# Autodesk Inventor assembly: AirtightAftSectionAssembly0
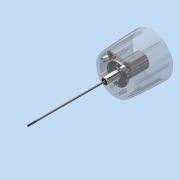
[picture p0: Inventor's stored thumbnail of the model, 180x180]
Saved by Autodesk Inventor 2017 (Build 210142000, 142)
## iProperties
Created: 2016-10-23
Part Number: AirtightAftSectionAssembly0
Document SubType Name: Assembly
Designer: techn
Author: techn
## Documents named in this file (6)
- D:\OneDrive\Documents\Other Projects\Submarine\CAD\aft\AirtightAftSectionAssembly0.iam
- D:\OneDrive\Documents\Other Projects\Submarine\CAD\aft\MotorAssembly0.iam
- D:\OneDrive\Documents\Other Projects\Submarine\CAD\aft\AftSectionAirtightRear.ipt
- D:\OneDrive\Documents\Other Projects\Submarine\CAD\common\PushRodSeal\Engel3mm\Engel3mmAssembly.iam
- D:\OneDrive\Documents\Other Projects\Submarine\CAD\common\PushRodSeal\bearingHousing.ipt
- D:\OneDrive\Documents\Other Projects\Submarine\CAD\common\SleeveBearing3mmFlanged.ipt
## Components (8 placed, 5 different names)
1. MotorAssembly0:1 [sub-assembly] — Mate:5, Mate:6, Mate:7
2. AftSectionAirtightRear:1 — Mate:5, Mate:6, Mate:7, Mate:23, Mate:24, Angle:1, Angle:2, Mate:25, Mate:26, Mate:33, Mate:34, Mate:35, Mate:36
3. Engel3mmAssembly:1 [sub-assembly] — Mate:23, Angle:2, Mate:25, Mate:31
4. Engel3mmAssembly:2 [sub-assembly] — Mate:24, Angle:1, Mate:26, Mate:32
5. bearingHousing:1 — Mate:27, Mate:28, Mate:33, Mate:34
6. bearingHousing:2 — Mate:29, Mate:30, Mate:31, Mate:35, Mate:36
7. SleeveBearing3mmFlanged:1 — Mate:27, Mate:28, Mate:32
8. SleeveBearing3mmFlanged:2 — Mate:29, Mate:30
## Relationships (19: Mate 17, Angle 2)
- Mate:5: MotorAssembly0:1 ↔ AftSectionAirtightRear:1
- Mate:6: MotorAssembly0:1 ↔ AftSectionAirtightRear:1
- Mate:7: MotorAssembly0:1 ↔ AftSectionAirtightRear:1
- Mate:23: AftSectionAirtightRear:1 ↔ Engel3mmAssembly:1
- Mate:24: AftSectionAirtightRear:1 ↔ Engel3mmAssembly:2
- Angle:1 (0 deg): AftSectionAirtightRear:1 ↔ Engel3mmAssembly:2
- Angle:2 (0 deg): AftSectionAirtightRear:1 ↔ Engel3mmAssembly:1
- Mate:25: AftSectionAirtightRear:1 ↔ Engel3mmAssembly:1
- Mate:26: AftSectionAirtightRear:1 ↔ Engel3mmAssembly:2
- Mate:27: bearingHousing:1 ↔ SleeveBearing3mmFlanged:1
- Mate:28: bearingHousing:1 ↔ SleeveBearing3mmFlanged:1
- Mate:29: bearingHousing:2 ↔ SleeveBearing3mmFlanged:2
- Mate:30: bearingHousing:2 ↔ SleeveBearing3mmFlanged:2
- Mate:31: Engel3mmAssembly:1 ↔ bearingHousing:2
- Mate:32: Engel3mmAssembly:2 ↔ SleeveBearing3mmFlanged:1
- Mate:33: AftSectionAirtightRear:1 ↔ bearingHousing:1
- Mate:34: AftSectionAirtightRear:1 ↔ bearingHousing:1
- Mate:35: AftSectionAirtightRear:1 ↔ bearingHousing:2
- Mate:36: AftSectionAirtightRear:1 ↔ bearingHousing:2
